# Autodesk Inventor assembly: armrest
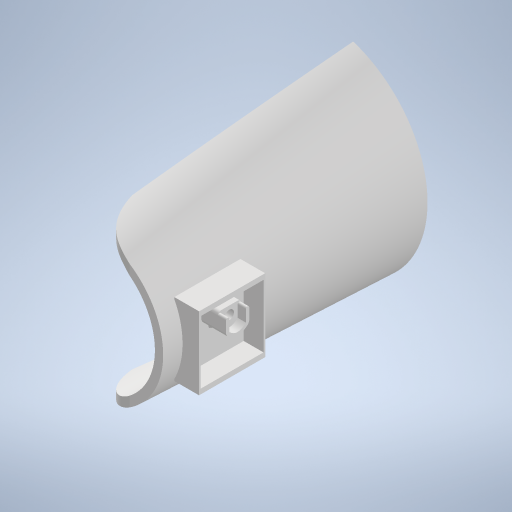
[picture p0: Inventor's stored thumbnail of the model, 512x512]
Saved by Autodesk Inventor 2024 (Build 280153000, 153)
## iProperties
Created: 2023-09-04
Part Number: armrest
Document SubType Name: Assembly
Designer: Pintu
Author: Pintu
## Documents named in this file (3)
- D:\CMC\my_inventor\ArmBo_v2\armrest.iam
- D:\CMC\my_inventor\ArmBo_v2\load_cell_holder.ipt
- D:\CMC\my_inventor\ArmBo_v2\cuff.ipt
## Components (2 placed, 2 different names)
1. load_cell_holder:1 — Mate:1
2. cuff:1 — Mate:1
## Relationships (1: Mate 1)
- Mate:1: load_cell_holder:1 ↔ cuff:1
